# Autodesk Inventor assembly: mid_brace
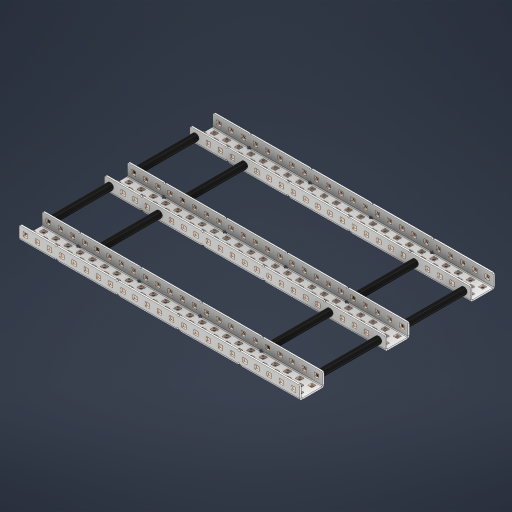
[picture p0: Inventor's stored thumbnail of the model, 512x512]
Saved by Autodesk Inventor 2024 (Build 280153000, 153)
## iProperties
Created: 2023-10-18
Part Number: mid_brace
Document SubType Name: Assembly
Designer: Averey Ku
Author: Averey Ku
## Documents named in this file (4)
- C:\Users\avere\Documents\rbp_cad\goated_v0.1\chassis\mid_brace.iam
- C:\Users\avere\Documents\rbp_cad\VEX-CAD-Inventor-1.41\Structure\C Channel\Aluminum 1x2x1\Alu C 1x2x1x23.ipt
- C:\Users\avere\Documents\rbp_cad\VEX-CAD-Inventor-1.41\Structure\Standoff\Standoff 2.50.ipt
- D:\vex_robotics\hardware\cad\VEX-CAD-Inventor-1.41\Structure\Standoff.ipt
## Components (11 placed, 2 different names)
1. Alu C 1x2x1x23:1 — Insert:1, Insert:3, Insert:4, Insert:5
2. Alu C 1x2x1x23:2 — Insert:2, Mate:1, Insert:6, Insert:7, Insert:8, Insert:9
3. Standoff 2.50:1 — Insert:1, Insert:2
4. Standoff 2.50:2 — Insert:3, Mate:1
5. Standoff 2.50:3 — Insert:4
6. Standoff 2.50:4 — Insert:5
7. Alu C 1x2x1x23:3 — Insert:10, Mate:2
8. Standoff 2.50:5 — Insert:6
9. Standoff 2.50:6 — Insert:7
10. Standoff 2.50:7 — Insert:8, Mate:2
11. Standoff 2.50:8 — Insert:9, Insert:10
## Relationships (12: Insert 10, Mate 2)
- Insert:1: Alu C 1x2x1x23:1 ↔ Standoff 2.50:1
- Insert:2: Alu C 1x2x1x23:2 ↔ Standoff 2.50:1
- Insert:3: Alu C 1x2x1x23:1 ↔ Standoff 2.50:2
- Mate:1: Alu C 1x2x1x23:2 ↔ Standoff 2.50:2
- Insert:4: Alu C 1x2x1x23:1 ↔ Standoff 2.50:3
- Insert:5: Alu C 1x2x1x23:1 ↔ Standoff 2.50:4
- Insert:6: Alu C 1x2x1x23:2 ↔ Standoff 2.50:5
- Insert:7: Alu C 1x2x1x23:2 ↔ Standoff 2.50:6
- Insert:8: Alu C 1x2x1x23:2 ↔ Standoff 2.50:7
- Insert:9: Alu C 1x2x1x23:2 ↔ Standoff 2.50:8
- Insert:10: Alu C 1x2x1x23:3 ↔ Standoff 2.50:8
- Mate:2: Alu C 1x2x1x23:3 ↔ Standoff 2.50:7
